# Autodesk Inventor assembly: Foot
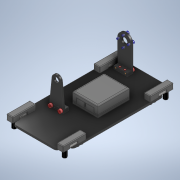
[picture p0: Inventor's stored thumbnail of the model, 180x180]
Saved by Autodesk Inventor 2022.3 (Build 263350000, 350)
## iProperties
Created: 2022-06-04
Part Number: Foot
Document SubType Name: Assembly
Designer: Masato Kubotera
Author: Masato Kubotera
## Documents named in this file (14)
- C:\Users\Masato\Documents\Inventor\Inventor for CIT Brains\SUSTAINA-OP - Foot\LowerBody\Foot\Foot.iam
- C:\Users\Masato\Documents\Inventor\Inventor for CIT Brains\SUSTAINA-OP - Foot\LowerBody\Foot\Foot_back_frame.ipt
- C:\Users\Masato\Documents\Inventor\Inventor for CIT Brains\SUSTAINA-OP - Foot\LowerBody\Foot\Foot_front_frame.ipt
- C:\Users\Masato\Documents\Inventor\Inventor for CIT Brains\SUSTAINA-OP - Foot\LowerBody\Foot\Foot_root_block.ipt
- C:\Users\Masato\Documents\Inventor\Inventor for CIT Brains\SUSTAINA-OP - Foot\LowerBody\Foot\Sole_frame.ipt
- C:\Users\Masato\Documents\Inventor\Inventor for CIT Brains\SUSTAINA-OP - Foot\ReadyMade\Screw\UC-0308.ipt
- C:\Users\Masato\Documents\Inventor\Inventor for CIT Brains\SUSTAINA-OP - Foot\ReadyMade\Screw\UC-2606.ipt
- C:\Users\Masato\Documents\Inventor\Inventor for CIT Brains\SUSTAINA-OP - Foot\ReadyMade\ElectronicComponents\Quad-Load-Cell-Amplifier-to-RS-485-Conv-Module.ipt
- C:\Users\Masato\Documents\Inventor\Inventor for CIT Brains\SUSTAINA-OP - Foot\LowerBody\Foot\Quad-Load-Cell-Amplifier-to-RS-485-Conv-Module-LowerCover.ipt
- C:\Users\Masato\Documents\Inventor\Inventor for CIT Brains\SUSTAINA-OP - Foot\LowerBody\Foot\Quad-Load-Cell-Amplifier-to-RS-485-Conv-Module-UpperCover.iam
- C:\Users\Masato\Documents\Inventor\Inventor for CIT Brains\SUSTAINA-OP - Foot\ReadyMade\Screw\UC-0310.ipt
- C:\Users\Masato\Documents\Inventor\Inventor for CIT Brains\SUSTAINA-OP - Foot\ReadyMade\ElectronicComponents\SC700-40kg.ipt
- C:\Users\Masato\Documents\Inventor\Inventor for CIT Brains\SUSTAINA-OP - Foot\ReadyMade\Spacer\ASL-312BE.ipt
- C:\Users\Masato\Documents\Inventor\Inventor for CIT Brains\SUSTAINA-OP - Foot\LowerBody\Foot\SC700-40kg_Cover.iam
## Components (48 placed, 13 different names)
1. Quad-Load-Cell-Amplifier-to-RS-485-Conv-Module:1 — 挿入:53, 挿入:54, 挿入:55, 挿入:56, 挿入:57, 挿入:58, 挿入:59, 挿入:60
2. Quad-Load-Cell-Amplifier-to-RS-485-Conv-Module-LowerCover:1 — 挿入:49, 挿入:50, 挿入:51, 挿入:52, 挿入:53, 挿入:54, 挿入:55, 挿入:56
3. Quad-Load-Cell-Amplifier-to-RS-485-Conv-Module-UpperCover:1 [sub-assembly] — 挿入:57, 挿入:58, 挿入:59, 挿入:60
4. SC700-40kg_Cover:1 [sub-assembly] — 挿入:89, 挿入:90
5. SC700-40kg_Cover:2 [sub-assembly] — 挿入:91, 挿入:94
6. SC700-40kg_Cover:3 [sub-assembly] — 挿入:92, 挿入:96
7. SC700-40kg_Cover:4 [sub-assembly] — 挿入:93, 挿入:95
8. Sole_frame:1 — 挿入:1, 挿入:2, 挿入:3, 挿入:4, 挿入:13, 挿入:14, 挿入:15, 挿入:16, 挿入:49, 挿入:50, 挿入:51, 挿入:52, 挿入:61, 挿入:62, 挿入:63, 挿入:64, 挿入:65, 挿入:66, 挿入:67, 挿入:68, 挿入:69, 挿入:70, 挿入:71, 挿入:72, 挿入:73, 挿入:74, 挿入:75, 挿入:76, 挿入:77, 挿入:78, 挿入:79, 挿入:80, フラッシュ:1, フラッシュ:2, フラッシュ:3
9. Foot_front_frame:1 — 挿入:5, 挿入:6, メイト:1, 挿入:31, 挿入:32
10. Foot_back_frame:1 — 挿入:7, 挿入:8, 挿入:17, 挿入:18, 挿入:19, 挿入:20, 挿入:29, 挿入:30
11. Foot_root_block:1 — 挿入:1, 挿入:2, 挿入:5, 挿入:6
12. Foot_root_block:2 — 挿入:3, 挿入:4, 挿入:7, 挿入:8
13. SC700-40kg:1 — 挿入:73, 挿入:74, 挿入:81, 挿入:85, 挿入:89, 挿入:90
14. SC700-40kg:2 — 挿入:75, 挿入:76, 挿入:82, 挿入:86, 挿入:91, 挿入:94
15. SC700-40kg:3 — 挿入:77, 挿入:78, 挿入:83, 挿入:87, 挿入:92, 挿入:96
16. SC700-40kg:4 — 挿入:79, 挿入:80, 挿入:84, 挿入:88, 挿入:93, 挿入:95
17. ASL-312BE:1 — 挿入:85
18. ASL-312BE:2 — 挿入:86
19. ASL-312BE:3 — 挿入:87
20. ASL-312BE:4 — 挿入:88
21. UC-0310:5 — 挿入:81
22. UC-0310:6 — 挿入:82
23. UC-0310:7 — 挿入:83
24. UC-0310:8 — 挿入:84
25. UC-0308:9 — 挿入:65
26. UC-0308:10 — 挿入:66
27. UC-0308:11 — 挿入:67
28. UC-0308:12 — 挿入:68
29. UC-0308:13 — 挿入:69
30. UC-0308:14 — 挿入:70
31. UC-0308:15 — 挿入:71
32. UC-0308:16 — 挿入:72
33. UC-0308:5 — 挿入:32
34. UC-0308:6 — 挿入:31
35. UC-0308:7 — 挿入:29
36. UC-0308:8 — 挿入:30
37. UC-0308:1 — 挿入:13
38. UC-0308:2 — 挿入:14
39. UC-0308:3 — 挿入:15
40. UC-0308:4 — 挿入:16
41. UC-2606:1 — 挿入:17
42. UC-2606:2 — 挿入:18
43. UC-2606:3 — 挿入:19
44. UC-2606:4 — 挿入:20
45. UC-0310:1 — 挿入:61
46. UC-0310:2 — 挿入:62
47. UC-0310:3 — 挿入:63
48. UC-0310:4 — 挿入:64
## Relationships (72: Insert 68, Flush 3, Mate 1)
- メイト:1 [Mate]: Foot_front_frame:1
- 挿入:1 [Insert]: Sole_frame:1 ↔ Foot_root_block:1
- 挿入:2 [Insert]: Sole_frame:1 ↔ Foot_root_block:1
- 挿入:3 [Insert]: Sole_frame:1 ↔ Foot_root_block:2
- 挿入:4 [Insert]: Sole_frame:1 ↔ Foot_root_block:2
- 挿入:5 [Insert]: Foot_front_frame:1 ↔ Foot_root_block:1
- 挿入:6 [Insert]: Foot_front_frame:1 ↔ Foot_root_block:1
- 挿入:7 [Insert]: Foot_back_frame:1 ↔ Foot_root_block:2
- 挿入:8 [Insert]: Foot_back_frame:1 ↔ Foot_root_block:2
- 挿入:13 [Insert]: Sole_frame:1 ↔ UC-0308:1
- 挿入:14 [Insert]: Sole_frame:1 ↔ UC-0308:2
- 挿入:15 [Insert]: Sole_frame:1 ↔ UC-0308:3
- 挿入:16 [Insert]: Sole_frame:1 ↔ UC-0308:4
- 挿入:17 [Insert]: Foot_back_frame:1 ↔ UC-2606:1
- 挿入:18 [Insert]: Foot_back_frame:1 ↔ UC-2606:2
- 挿入:19 [Insert]: Foot_back_frame:1 ↔ UC-2606:3
- 挿入:20 [Insert]: Foot_back_frame:1 ↔ UC-2606:4
- 挿入:29 [Insert]: Foot_back_frame:1 ↔ UC-0308:7
- 挿入:30 [Insert]: Foot_back_frame:1 ↔ UC-0308:8
- 挿入:31 [Insert]: Foot_front_frame:1 ↔ UC-0308:6
- 挿入:32 [Insert]: Foot_front_frame:1 ↔ UC-0308:5
- 挿入:49 [Insert]: Quad-Load-Cell-Amplifier-to-RS-485-Conv-Module-LowerCover:1 ↔ Sole_frame:1
- 挿入:50 [Insert]: Quad-Load-Cell-Amplifier-to-RS-485-Conv-Module-LowerCover:1 ↔ Sole_frame:1
- 挿入:51 [Insert]: Quad-Load-Cell-Amplifier-to-RS-485-Conv-Module-LowerCover:1 ↔ Sole_frame:1
- 挿入:52 [Insert]: Quad-Load-Cell-Amplifier-to-RS-485-Conv-Module-LowerCover:1 ↔ Sole_frame:1
- 挿入:53 [Insert]: Quad-Load-Cell-Amplifier-to-RS-485-Conv-Module:1 ↔ Quad-Load-Cell-Amplifier-to-RS-485-Conv-Module-LowerCover:1
- 挿入:54 [Insert]: Quad-Load-Cell-Amplifier-to-RS-485-Conv-Module:1 ↔ Quad-Load-Cell-Amplifier-to-RS-485-Conv-Module-LowerCover:1
- 挿入:55 [Insert]: Quad-Load-Cell-Amplifier-to-RS-485-Conv-Module:1 ↔ Quad-Load-Cell-Amplifier-to-RS-485-Conv-Module-LowerCover:1
- 挿入:56 [Insert]: Quad-Load-Cell-Amplifier-to-RS-485-Conv-Module:1 ↔ Quad-Load-Cell-Amplifier-to-RS-485-Conv-Module-LowerCover:1
- 挿入:57 [Insert]: Quad-Load-Cell-Amplifier-to-RS-485-Conv-Module:1 ↔ Quad-Load-Cell-Amplifier-to-RS-485-Conv-Module-UpperCover:1
- 挿入:58 [Insert]: Quad-Load-Cell-Amplifier-to-RS-485-Conv-Module:1 ↔ Quad-Load-Cell-Amplifier-to-RS-485-Conv-Module-UpperCover:1
- 挿入:59 [Insert]: Quad-Load-Cell-Amplifier-to-RS-485-Conv-Module:1 ↔ Quad-Load-Cell-Amplifier-to-RS-485-Conv-Module-UpperCover:1
- 挿入:60 [Insert]: Quad-Load-Cell-Amplifier-to-RS-485-Conv-Module:1 ↔ Quad-Load-Cell-Amplifier-to-RS-485-Conv-Module-UpperCover:1
- 挿入:61 [Insert]: Sole_frame:1 ↔ UC-0310:1
- 挿入:62 [Insert]: Sole_frame:1 ↔ UC-0310:2
- 挿入:63 [Insert]: Sole_frame:1 ↔ UC-0310:3
- 挿入:64 [Insert]: Sole_frame:1 ↔ UC-0310:4
- 挿入:65 [Insert]: Sole_frame:1 ↔ UC-0308:9
- 挿入:66 [Insert]: Sole_frame:1 ↔ UC-0308:10
- 挿入:67 [Insert]: Sole_frame:1 ↔ UC-0308:11
- 挿入:68 [Insert]: Sole_frame:1 ↔ UC-0308:12
- 挿入:69 [Insert]: Sole_frame:1 ↔ UC-0308:13
- 挿入:70 [Insert]: Sole_frame:1 ↔ UC-0308:14
- 挿入:71 [Insert]: Sole_frame:1 ↔ UC-0308:15
- 挿入:72 [Insert]: Sole_frame:1 ↔ UC-0308:16
- 挿入:73 [Insert]: Sole_frame:1 ↔ SC700-40kg:1
- 挿入:74 [Insert]: Sole_frame:1 ↔ SC700-40kg:1
- 挿入:75 [Insert]: Sole_frame:1 ↔ SC700-40kg:2
- 挿入:76 [Insert]: Sole_frame:1 ↔ SC700-40kg:2
- 挿入:77 [Insert]: Sole_frame:1 ↔ SC700-40kg:3
- 挿入:78 [Insert]: Sole_frame:1 ↔ SC700-40kg:3
- 挿入:79 [Insert]: Sole_frame:1 ↔ SC700-40kg:4
- 挿入:80 [Insert]: Sole_frame:1 ↔ SC700-40kg:4
- 挿入:81 [Insert]: SC700-40kg:1 ↔ UC-0310:5
- 挿入:82 [Insert]: SC700-40kg:2 ↔ UC-0310:6
- 挿入:83 [Insert]: SC700-40kg:3 ↔ UC-0310:7
- 挿入:84 [Insert]: SC700-40kg:4 ↔ UC-0310:8
- 挿入:85 [Insert]: SC700-40kg:1 ↔ ASL-312BE:1
- 挿入:86 [Insert]: SC700-40kg:2 ↔ ASL-312BE:2
- 挿入:87 [Insert]: SC700-40kg:3 ↔ ASL-312BE:3
- 挿入:88 [Insert]: SC700-40kg:4 ↔ ASL-312BE:4
- 挿入:89 [Insert]: SC700-40kg_Cover:1 ↔ SC700-40kg:1
- フラッシュ:1 [Flush]: Sole_frame:1
- フラッシュ:2 [Flush]: Sole_frame:1
- フラッシュ:3 [Flush]: Sole_frame:1
- 挿入:90 [Insert]: SC700-40kg_Cover:1 ↔ SC700-40kg:1
- 挿入:91 [Insert]: SC700-40kg_Cover:2 ↔ SC700-40kg:2
- 挿入:92 [Insert]: SC700-40kg_Cover:3 ↔ SC700-40kg:3
- 挿入:93 [Insert]: SC700-40kg_Cover:4 ↔ SC700-40kg:4
- 挿入:94 [Insert]: SC700-40kg_Cover:2 ↔ SC700-40kg:2
- 挿入:95 [Insert]: SC700-40kg_Cover:4 ↔ SC700-40kg:4
- 挿入:96 [Insert]: SC700-40kg_Cover:3 ↔ SC700-40kg:3
